# Autodesk Inventor assembly: Full_SigmaBan_106AT_nuc
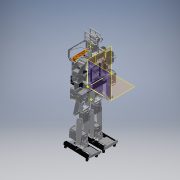
[picture p0: Inventor's stored thumbnail of the model, 180x180]
Saved by Autodesk Inventor 2018 (Build 220112000, 112)
## iProperties
Created: 2017-01-31
Part Number: Full_SigmaBan_106AT_nuc
Document SubType Name: Assembly
Designer: steve
Mass: 4494.03 g
Surface Area: 10713.9 cm^2
Volume: 2303.92 cm^3
Density: 1.9506 g/cm^3
Author: steve
## Documents named in this file (44)
- C:\Users\patxi\Dropbox\SigmaBan\SigmaBanV2.1\Full_SigmaBan_106AT_nuc.iam
- C:\Users\patxi\Dropbox\SigmaBan\SigmaBanV2.1\SigmaBan_torsebas64.ipt
- C:\Users\patxi\Dropbox\SigmaBan\SigmaBanV2.1\battery.ipt
- C:\Users\patxi\Dropbox\SigmaBan\SigmaBanV2.1\backboard.ipt
- C:\Users\patxi\Dropbox\SigmaBan\SigmaBanV2.1\newhub.ipt
- C:\Users\patxi\Dropbox\SigmaBan\SigmaBanV2.1\MX-64AT_AR_sideR.iam
- C:\Users\patxi\Dropbox\SigmaBan\SigmaBanV2.1\MX-64AT_AR_sideL.iam
- C:\Users\patxi\Dropbox\SigmaBan\SigmaBanV2.1\bloc_double106.iam
- C:\Users\patxi\Dropbox\SigmaBan\SigmaBanV2.1\MX-106T_bottom.iam
- C:\Users\patxi\Dropbox\SigmaBan\SigmaBanV2.1\Sigma106_tibiaplate_design.ipt
- C:\Users\patxi\Dropbox\SigmaBan\SigmaBanV2.1\MX-64AT_AR_contreaxe.iam
- C:\Users\patxi\Dropbox\SigmaBan\SigmaBanV2.1\beeper.ipt
- C:\Users\patxi\Dropbox\SigmaBan\SigmaBanV2.1\pillar_tube.ipt
- C:\Users\patxi\Dropbox\SigmaBan\SigmaBanV2.1\fitplate.ipt
- C:\Users\patxi\Dropbox\SigmaBan\SigmaBanV2.1\new_torso_topplate_nuc.ipt
- C:\Users\patxi\Dropbox\SigmaBan\SigmaBanV2.1\new_torso_middleplate_nuc.ipt
- C:\Users\patxi\Dropbox\SigmaBan\SigmaBanV2.1\Intel NUC6i3SYK.ipt
- C:\Users\patxi\Dropbox\SigmaBan\SigmaBanV2.1\new_U\new_u64_2.iam
- C:\Users\patxi\Dropbox\SigmaBan\SigmaBanV2.1\Ulong\u106_long_design_newbearing.iam
- C:\Users\patxi\Dropbox\SigmaBan\SigmaBanV2.1\piano_wire_protection.ipt
- C:\Users\patxi\Dropbox\SigmaBan\SigmaBanV2.1\high_leg_teflon_left.ipt
- C:\Users\patxi\Dropbox\SigmaBan\SigmaBanV2.1\high_leg_teflon_right.ipt
- C:\Users\patxi\Dropbox\SigmaBan\SigmaBanV2.1\new_U\new_U64_shoulder_with_offset.iam
- C:\Users\patxi\Dropbox\SigmaBan\SigmaBanV2.1\humerus.ipt
- C:\Users\patxi\Dropbox\SigmaBan\SigmaBanV2.1\FR05-H101.ipt
- C:\Users\patxi\Dropbox\SigmaBan\SigmaBanV2.1\FR05-S101.ipt
- C:\Users\patxi\Dropbox\SigmaBan\SigmaBanV2.1\radius.ipt
- C:\Users\patxi\Dropbox\SigmaBan\SigmaBanV2.1\elbow_protection.ipt
- C:\Users\patxi\Dropbox\SigmaBan\SigmaBanV2.1\new_u64_shoulder.iam
- C:\Users\patxi\Dropbox\SigmaBan\SigmaBanV2.1\head_mx64\head_assembly.iam
- C:\Users\patxi\Dropbox\SigmaBan\SigmaBanV2.1\nuc_fix_v2.ipt
- C:\Users\patxi\Dropbox\SigmaBan\SigmaBanV2.1\piano_wire_back_fixation.ipt
- C:\Users\patxi\Dropbox\SigmaBan\SigmaBanV2.1\back_piano_wire.ipt
- C:\Users\patxi\Dropbox\SigmaBan\SigmaBanV2.1\shoulder_piano_wire_fix.ipt
- C:\Users\patxi\Dropbox\SigmaBan\SigmaBanV2.1\shoulder_piano wire.ipt
- C:\Users\patxi\Dropbox\SigmaBan\SigmaBanV2.1\foot_with_cleat.iam
- C:\Users\patxi\Dropbox\SigmaBan\SigmaBanV2.1\bloc_double106_MIR.iam
- C:\Users\patxi\Dropbox\SigmaBan\SigmaBanV2.1\dynamixel\frames\FR08-B101.ipt
- C:\Users\patxi\Dropbox\SigmaBan\SigmaBanV2.1\MX-64AT_AR.ipt
- C:\Users\patxi\Dropbox\SigmaBan\SigmaBanV2.1\dynamixel\motors\mx106-contre-axe.iam
- C:\Users\patxi\Dropbox\SigmaBan\SigmaBanV2.1\low_torso_protection.ipt
- C:\Users\patxi\Dropbox\SigmaBan\SigmaBanV2.1\high_torso_protection.ipt
- C:\Users\patxi\Dropbox\SigmaBan\SigmaBanV2.1\external\M3_cube_standoff.ipt
- C:\Users\patxi\Dropbox\SigmaBan\SigmaBanV2.1\handle_v3.ipt
## Components (80 placed, 49 different names)
1. SigmaBan_torsebas64:1 — Mate:98, Flush:8, Flush:9, Mate:548, Mate:551, Mate:552, Mate:553
2. FR08-B101:1 — Mate:442, Mate:443, Mate:481, Mate:482, Mate:483
3. FR08-B101:2 — Mate:446, Mate:447, Mate:448, Mate:473, Mate:474, Mate:475
4. battery:1 — Mate:98, Flush:8, Flush:9
5. new_torso_topplate_nuc:1 — Mate:57, Mate:58, Mate:59, Mate:60, Mate:61, Mate:62, Mate:233, Mate:234, Mate:235, Mate:248, Mate:249, Mate:251, Flush:3, Mate:252, Mate:271, Flush:5, Mate:391, Mate:392, Mate:453, Mate:456, Flush:11, Mate:555, Flush:12, Mate:556, Mate:560, Mate:561, Mate:562, Mate:564, Mate:565, Mate:566
6. new_torso_middleplate_nuc:1 — Mate:214, Mate:215, Mate:236, Mate:239, Mate:240, Mate:241, Mate:242, Mate:256, Mate:257, Mate:258, Mate:259, Flush:4, Mate:442, Mate:443, Mate:446, Mate:447, Mate:448, Mate:550, Mate:554
7. Motor:right_shoulder_pitch [sub-assembly] — Mate:57, Mate:59, Mate:60, Mate:349, Mate:350
8. Motor:left_shoulder_pitch [sub-assembly] — Mate:58, Mate:61, Mate:62, Mate:345, Mate:346, DOF:left_shoulder_pitch
9. Motor:right_hip_pitch — Mate:473, Mate:474, Mate:475, Mate:476, Mate:477, Mate:478, Mate:479, Mate:480, Mate:551, Mate:552, Mate:553
10. Motor:left_hip [sub-assembly] — Mate:141, Mate:282, Mate:428, Mate:539, Mate:540, DOF:left_hip_pitch, DOF:left_hip_yaw, DOF:left_hip_roll
11. Motor:right_hip [sub-assembly] — Mate:278, Mate:435, Mate:541, Mate:542
12. Motor:left_knee [sub-assembly] — Mate:150, Mate:164, Mate:287, DOF:left_hip_pitch, DOF:left_knee, Mate:429, Mate:430, Mate:431, Mate:432
13. Motor:left_ankle [sub-assembly] — Mate:143, Mate:151, Mate:162, Mate:163, DOF:left_ankle_pitch, Mate:543, Mate:544
14. Motor:right_ankle [sub-assembly] — DOF:right_ankle_pitch, Mate:433, Mate:434, Mate:439, Mate:545, Mate:546
15. Sigma106_tibiaplate_design:1 — Mate:150, Mate:151, DOF:left_knee, DOF:left_ankle_pitch, Mate:432
16. Sigma106_tibiaplate_design:2 — DOF:right_ankle_pitch, Mate:433, Mate:434, Mate:464, Mate:466
17. Sigma106_tibiaplate_design:3 — Mate:439, Mate:465, Mate:547
18. Sigma106_tibiaplate_design:4 — Mate:162, Mate:163, Mate:164, Mate:431
19. u106_long_design_newbearing:1 [sub-assembly] — Mate:282, Mate:287, Mate:428, Mate:429, Mate:430
20. u106_long_design_newbearing:2 [sub-assembly] — Mate:278, Mate:435, Mate:470, Mate:471, Mate:472
21. new_u64_2:2 [sub-assembly] — Mate:484, Mate:485, Mate:539, Mate:540
22. new_u64_2:3 [sub-assembly] — Mate:416, Mate:417, Mate:418, Mate:543, Mate:544
23. new_u64_2:4 [sub-assembly] — Mate:476, Mate:477, Mate:541, Mate:542
24. new_u64_2:5 [sub-assembly] — Mate:421, Mate:422, Mate:423, Mate:545, Mate:546
25. Motor:left_shoulder_roll [sub-assembly] — Mate:347, Mate:348, Mate:404, Mate:405, Mate:406, Mate:407, Mate:408, Mate:409, DOF:left_shoulder_roll, Mate:491, Mate:492, Mate:493
26. newhub:2 — Mate:214, Mate:215, Mate:441, Flush:10
27. backboard:3 — Mate:233, Mate:234, Mate:235
28. beeper:1 — Mate:236, Mate:441, Flush:10
29. pillar_tube:1 — Mate:239, Mate:248, Mate:256
30. pillar_tube:2 — Mate:240, Mate:249, Mate:259
31. pillar_tube:3 — Mate:242, Mate:258, Mate:390
32. pillar_tube:4 — Mate:241, Mate:257, Mate:271
33. fitplate:1 — Mate:251, Flush:3, Mate:252
34. MX-64AT_AR_contreaxe:2 [sub-assembly] — Mate:351, Mate:352, Angle:29, Mate:503, Mate:504, Mate:505, Mate:534, Mate:535, Mate:536
35. Intel NUC6i3SYK:1 — Flush:4, Flush:5, Flush:11
36. FR08-B101:3 — Mate:453, Mate:456, Mate:458, Mate:460, Mate:461
37. piano_wire_protection:1 — Mate:563, Mate:567
38. high_leg_teflon_left:1 — Mate:486, Mate:487, Mate:488
39. high_leg_teflon_right:1 — Mate:478, Mate:479, Mate:480
40. new_U64_shoulder_with_offset:1 [sub-assembly] — Mate:345, Mate:346, Mate:347, Mate:348, DOF:left_shoulder_pitch, DOF:left_shoulder_roll
41. new_U64_shoulder_with_offset:2 [sub-assembly] — Mate:349, Mate:350, Mate:351, Mate:352, Angle:29
42. humerus:1 — Mate:372, Mate:373, Mate:374, DOF:left_elbow, Mate:494, Mate:495, Mate:496
43. humerus:2 — Mate:506, Mate:507, Mate:508, Mate:519, Mate:520, Mate:521
44. FR05-H101:1 — Mate:372, Mate:373, Mate:374, Mate:375, Mate:376, Mate:383, Mate:384, Mate:385
45. Motor:left_elbow [sub-assembly] — Mate:375, Mate:376, DOF:left_elbow, Mate:497, Mate:498, Mate:499
46. FR05-S101:1 — Mate:497, Mate:498, Mate:499, Mate:500, Mate:501, Mate:502
47. radius:1 — Mate:500, Mate:501, Mate:502
48. elbow_protection:1 — Mate:383, Mate:384, Mate:385
49. new_u64_shoulder:1 [sub-assembly] — DOF:head_pitch, Mate:413, Mate:414, Mate:457, Mate:459
50. head_assembly:1 [sub-assembly] — DOF:head_pitch, Mate:413, Mate:414, DOF:head_yaw
51. nuc_fix_v2:1 — Mate:390, Mate:391, Mate:392, Mate:393, Mate:394, Mate:395, Mate:396, Mate:397, Mate:398
52. piano_wire_back_fixation:1 — Mate:393, Mate:394, Mate:395, Mate:400, Mate:570, Mate:571
53. piano_wire_back_fixation:2 — Mate:396, Mate:397, Mate:398, Mate:399, Mate:401, Mate:568, Mate:569
54. back_piano_wire:1 — Mate:399, Mate:400, Mate:401
55. shoulder_piano_wire_fix:1 — Mate:404, Mate:405, Mate:406, Mate:411, Mate:412
56. shoulder_piano_wire_fix:2 — Mate:407, Mate:408, Mate:409, Mate:410
57. shoulder_piano wire:1 — Mate:410, Mate:411, Mate:412
58. foot_with_cleat:1 [sub-assembly] — Mate:416, Mate:417, Mate:418
59. foot_with_cleat:2 [sub-assembly] — Mate:421, Mate:422, Mate:423
60. Motor:head_yaw — Mate:457, Mate:458, Mate:459, Mate:460, Mate:461, DOF:head_yaw, Flush:13
61. mx106-contre-axe:1 [sub-assembly] — Mate:464, Mate:465, Mate:466, Mate:467, Mate:468, Mate:469, Mate:547
62. FR05-S101:2 — Mate:467, Mate:468, Mate:469, Mate:470, Mate:471, Mate:472
63. Motor:left_hip_yaw — Mate:481, Mate:482, Mate:483, Mate:484, Mate:485, Mate:486, Mate:487, Mate:488, DOF:left_hip_yaw, DOF:left_hip_roll
64. FR05-S101:3 — Mate:491, Mate:492, Mate:493, Mate:494, Mate:495, Mate:496
65. FR05-S101:4 — Mate:503, Mate:504, Mate:505, Mate:506, Mate:507, Mate:508
66. FR05-H101:2 — Mate:517, Mate:518, Mate:519, Mate:520, Mate:521, Mate:525, Mate:526, Mate:527
67. MX-64AT_AR_contreaxe:4 [sub-assembly] — Mate:517, Mate:518, Mate:522, Mate:523, Mate:524
68. FR05-S101:5 — Mate:522, Mate:523, Mate:524
69. radius:2
70. elbow_protection:2 — Mate:525, Mate:526, Mate:527
71. shoulder_piano_wire_fix:3 — Mate:532, Mate:533, Mate:534, Mate:535, Mate:536
72. shoulder_piano_wire_fix:4 — Mate:537, Mate:538
73. shoulder_piano wire:2 — Mate:532, Mate:533, Mate:537, Mate:538
74. low_torso_protection:1 — Mate:548, Mate:550, Mate:554
75. high_torso_protection:1 — Mate:555, Flush:12, Mate:556
76. piano_wire_back_fixation:3 — Mate:560, Mate:561, Mate:562, Mate:563, Mate:567
77. piano_wire_back_fixation:4 — Mate:564, Mate:565, Mate:566
78. M3_cube_standoff:1 — Mate:570, Mate:571, Mate:574
79. M3_cube_standoff:2 — Mate:568, Mate:569, Mate:572, Mate:573
80. handle_v3:1 — Mate:572, Mate:573, Mate:574
## Relationships (222: Mate 201, Angle 12, Flush 9)
- Mate:57: new_torso_topplate_nuc:1 ↔ Motor:right_shoulder_pitch
- Mate:58: new_torso_topplate_nuc:1 ↔ Motor:left_shoulder_pitch
- Mate:59: new_torso_topplate_nuc:1 ↔ Motor:right_shoulder_pitch
- Mate:60: new_torso_topplate_nuc:1 ↔ Motor:right_shoulder_pitch
- Mate:61: new_torso_topplate_nuc:1 ↔ Motor:left_shoulder_pitch
- Mate:62: new_torso_topplate_nuc:1 ↔ Motor:left_shoulder_pitch
- [Mate]: FR08-B101:1 ↔ new_torso_middleplate_nuc:1
- Mate:98: SigmaBan_torsebas64:1 ↔ battery:1
- Mate:141: Motor:left_hip
- Mate:143: Motor:left_ankle
- Mate:150: Motor:left_knee ↔ Sigma106_tibiaplate_design:1
- Mate:151: Motor:left_ankle ↔ Sigma106_tibiaplate_design:1
- Mate:162: Motor:left_ankle ↔ Sigma106_tibiaplate_design:4
- Mate:163: Motor:left_ankle ↔ Sigma106_tibiaplate_design:4
- Mate:164: Motor:left_knee ↔ Sigma106_tibiaplate_design:4
- Mate:214: new_torso_middleplate_nuc:1 ↔ newhub:2
- Mate:215: new_torso_middleplate_nuc:1 ↔ newhub:2
- Mate:233: new_torso_topplate_nuc:1 ↔ backboard:3
- Mate:234: new_torso_topplate_nuc:1 ↔ backboard:3
- Mate:235: new_torso_topplate_nuc:1 ↔ backboard:3
- Mate:236: new_torso_middleplate_nuc:1 ↔ beeper:1
- Mate:239: new_torso_middleplate_nuc:1 ↔ pillar_tube:1
- Mate:240: new_torso_middleplate_nuc:1 ↔ pillar_tube:2
- Mate:241: new_torso_middleplate_nuc:1 ↔ pillar_tube:4
- Mate:242: new_torso_middleplate_nuc:1 ↔ pillar_tube:3
- Mate:248: new_torso_topplate_nuc:1 ↔ pillar_tube:1
- Mate:249: new_torso_topplate_nuc:1 ↔ pillar_tube:2
- Mate:251: new_torso_topplate_nuc:1 ↔ fitplate:1
- Flush:3: new_torso_topplate_nuc:1 ↔ fitplate:1
- Mate:252: new_torso_topplate_nuc:1 ↔ fitplate:1
- Mate:256: new_torso_middleplate_nuc:1 ↔ pillar_tube:1
- Mate:257: new_torso_middleplate_nuc:1 ↔ pillar_tube:4
- Mate:258: new_torso_middleplate_nuc:1 ↔ pillar_tube:3
- Mate:259: new_torso_middleplate_nuc:1 ↔ pillar_tube:2
- Mate:271: new_torso_topplate_nuc:1 ↔ pillar_tube:4
- Flush:4: new_torso_middleplate_nuc:1 ↔ Intel NUC6i3SYK:1
- Flush:5: new_torso_topplate_nuc:1 ↔ Intel NUC6i3SYK:1
- Mate:278: Motor:right_hip ↔ u106_long_design_newbearing:2
- Mate:282: Motor:left_hip ↔ u106_long_design_newbearing:1
- Mate:287: Motor:left_knee ↔ u106_long_design_newbearing:1
- [Mate]: new_torso_topplate_nuc:1 ↔ FR08-B101:3
- Flush:8: SigmaBan_torsebas64:1 ↔ battery:1
- Flush:9: SigmaBan_torsebas64:1 ↔ battery:1
- Mate:345: Motor:left_shoulder_pitch ↔ new_U64_shoulder_with_offset:1
- Mate:346: Motor:left_shoulder_pitch ↔ new_U64_shoulder_with_offset:1
- Mate:347: Motor:left_shoulder_roll ↔ new_U64_shoulder_with_offset:1
- Mate:348: Motor:left_shoulder_roll ↔ new_U64_shoulder_with_offset:1
- Mate:349: Motor:right_shoulder_pitch ↔ new_U64_shoulder_with_offset:2
- Mate:350: Motor:right_shoulder_pitch ↔ new_U64_shoulder_with_offset:2
- Mate:351: MX-64AT_AR_contreaxe:2 ↔ new_U64_shoulder_with_offset:2
- Mate:352: MX-64AT_AR_contreaxe:2 ↔ new_U64_shoulder_with_offset:2
- Angle:29 (0 deg): MX-64AT_AR_contreaxe:2 ↔ new_U64_shoulder_with_offset:2
- Mate:372: humerus:1 ↔ FR05-H101:1
- Mate:373: humerus:1 ↔ FR05-H101:1
- Mate:374: humerus:1 ↔ FR05-H101:1
- Mate:375: FR05-H101:1 ↔ Motor:left_elbow
- Mate:376: FR05-H101:1 ↔ Motor:left_elbow
- DOF:left_elbow [Angle] (0 deg): humerus:1 ↔ Motor:left_elbow
- Mate:383: FR05-H101:1 ↔ elbow_protection:1
- Mate:384: FR05-H101:1 ↔ elbow_protection:1
- Mate:385: FR05-H101:1 ↔ elbow_protection:1
- DOF:head_pitch [Angle] (0 deg): new_u64_shoulder:1 ↔ head_assembly:1
- Mate:390: pillar_tube:3 ↔ nuc_fix_v2:1
- Mate:391: new_torso_topplate_nuc:1 ↔ nuc_fix_v2:1
- Mate:392: new_torso_topplate_nuc:1 ↔ nuc_fix_v2:1
- Mate:393: nuc_fix_v2:1 ↔ piano_wire_back_fixation:1
- Mate:394: nuc_fix_v2:1 ↔ piano_wire_back_fixation:1
- Mate:395: nuc_fix_v2:1 ↔ piano_wire_back_fixation:1
- Mate:396: nuc_fix_v2:1 ↔ piano_wire_back_fixation:2
- Mate:397: nuc_fix_v2:1 ↔ piano_wire_back_fixation:2
- Mate:398: nuc_fix_v2:1 ↔ piano_wire_back_fixation:2
- Mate:399: piano_wire_back_fixation:2 ↔ back_piano_wire:1
- Mate:400: piano_wire_back_fixation:1 ↔ back_piano_wire:1
- Mate:401: piano_wire_back_fixation:2 ↔ back_piano_wire:1
- Mate:404: Motor:left_shoulder_roll ↔ shoulder_piano_wire_fix:1
- Mate:405: Motor:left_shoulder_roll ↔ shoulder_piano_wire_fix:1
- Mate:406: Motor:left_shoulder_roll ↔ shoulder_piano_wire_fix:1
- Mate:407: Motor:left_shoulder_roll ↔ shoulder_piano_wire_fix:2
- Mate:408: Motor:left_shoulder_roll ↔ shoulder_piano_wire_fix:2
- Mate:409: Motor:left_shoulder_roll ↔ shoulder_piano_wire_fix:2
- Mate:410: shoulder_piano_wire_fix:2 ↔ shoulder_piano wire:1
- Mate:411: shoulder_piano_wire_fix:1 ↔ shoulder_piano wire:1
- Mate:412: shoulder_piano_wire_fix:1 ↔ shoulder_piano wire:1
- Mate:413: new_u64_shoulder:1 ↔ head_assembly:1
- Mate:414: new_u64_shoulder:1 ↔ head_assembly:1
- DOF:left_hip_pitch [Angle] (0 deg): Motor:left_hip ↔ Motor:left_knee
- DOF:left_knee [Angle] (0 deg): Motor:left_knee ↔ Sigma106_tibiaplate_design:1
- DOF:left_ankle_pitch [Angle] (0 deg): Motor:left_ankle ↔ Sigma106_tibiaplate_design:1
- DOF:left_shoulder_pitch [Angle] (0 deg): Motor:left_shoulder_pitch ↔ new_U64_shoulder_with_offset:1
- DOF:left_shoulder_roll [Angle] (0 deg): Motor:left_shoulder_roll ↔ new_U64_shoulder_with_offset:1
- Mate:416: new_u64_2:3 ↔ foot_with_cleat:1
- Mate:417: new_u64_2:3 ↔ foot_with_cleat:1
- Mate:418: new_u64_2:3 ↔ foot_with_cleat:1
- Mate:421: new_u64_2:5 ↔ foot_with_cleat:2
- Mate:422: new_u64_2:5 ↔ foot_with_cleat:2
- DOF:right_ankle_pitch [Angle] (0 deg): Motor:right_ankle ↔ Sigma106_tibiaplate_design:2
- Mate:423: new_u64_2:5 ↔ foot_with_cleat:2
- Mate:428: Motor:left_hip ↔ u106_long_design_newbearing:1
- Mate:429: Motor:left_knee ↔ u106_long_design_newbearing:1
- Mate:430: Motor:left_knee ↔ u106_long_design_newbearing:1
- Mate:431: Motor:left_knee ↔ Sigma106_tibiaplate_design:4
- Mate:432: Motor:left_knee ↔ Sigma106_tibiaplate_design:1
- Mate:433: Motor:right_ankle ↔ Sigma106_tibiaplate_design:2
- Mate:434: Motor:right_ankle ↔ Sigma106_tibiaplate_design:2
- Mate:435: Motor:right_hip ↔ u106_long_design_newbearing:2
- Mate:439: Motor:right_ankle ↔ Sigma106_tibiaplate_design:3
- Mate:441: newhub:2 ↔ beeper:1
- Flush:10: newhub:2 ↔ beeper:1
- Mate:442: FR08-B101:1 ↔ new_torso_middleplate_nuc:1
- Mate:443: FR08-B101:1 ↔ new_torso_middleplate_nuc:1
- Mate:446: FR08-B101:2 ↔ new_torso_middleplate_nuc:1
- Mate:447: FR08-B101:2 ↔ new_torso_middleplate_nuc:1
- Mate:448: FR08-B101:2 ↔ new_torso_middleplate_nuc:1
- Mate:453: new_torso_topplate_nuc:1 ↔ FR08-B101:3
- Mate:456: new_torso_topplate_nuc:1 ↔ FR08-B101:3
- Mate:457: new_u64_shoulder:1 ↔ Motor:head_yaw
- Mate:458: FR08-B101:3 ↔ Motor:head_yaw
- Mate:459: new_u64_shoulder:1 ↔ Motor:head_yaw
- Mate:460: FR08-B101:3 ↔ Motor:head_yaw
- Mate:461: FR08-B101:3 ↔ Motor:head_yaw
- Mate:464: Sigma106_tibiaplate_design:2 ↔ mx106-contre-axe:1
- Mate:465: Sigma106_tibiaplate_design:3 ↔ mx106-contre-axe:1
- Mate:466: Sigma106_tibiaplate_design:2 ↔ mx106-contre-axe:1
- Mate:467: mx106-contre-axe:1 ↔ FR05-S101:2
- Mate:468: mx106-contre-axe:1 ↔ FR05-S101:2
- Mate:469: mx106-contre-axe:1 ↔ FR05-S101:2
- Mate:470: u106_long_design_newbearing:2 ↔ FR05-S101:2
- Mate:471: u106_long_design_newbearing:2 ↔ FR05-S101:2
- Mate:472: u106_long_design_newbearing:2 ↔ FR05-S101:2
- Mate:473: FR08-B101:2 ↔ Motor:right_hip_pitch
- Mate:474: FR08-B101:2 ↔ Motor:right_hip_pitch
- Mate:475: FR08-B101:2 ↔ Motor:right_hip_pitch
- Mate:476: Motor:right_hip_pitch ↔ new_u64_2:4
- Mate:477: Motor:right_hip_pitch ↔ new_u64_2:4
- Mate:478: Motor:right_hip_pitch ↔ high_leg_teflon_right:1
- Mate:479: Motor:right_hip_pitch ↔ high_leg_teflon_right:1
- Mate:480: Motor:right_hip_pitch ↔ high_leg_teflon_right:1
- Mate:481: FR08-B101:1 ↔ Motor:left_hip_yaw
- Mate:482: FR08-B101:1 ↔ Motor:left_hip_yaw
- Mate:483: FR08-B101:1 ↔ Motor:left_hip_yaw
- Mate:484: new_u64_2:2 ↔ Motor:left_hip_yaw
- Mate:485: new_u64_2:2 ↔ Motor:left_hip_yaw
- Mate:486: high_leg_teflon_left:1 ↔ Motor:left_hip_yaw
- Mate:487: high_leg_teflon_left:1 ↔ Motor:left_hip_yaw
- Mate:488: high_leg_teflon_left:1 ↔ Motor:left_hip_yaw
- Mate:491: Motor:left_shoulder_roll ↔ FR05-S101:3
- Mate:492: Motor:left_shoulder_roll ↔ FR05-S101:3
- Mate:493: Motor:left_shoulder_roll ↔ FR05-S101:3
- Mate:494: humerus:1 ↔ FR05-S101:3
- Mate:495: humerus:1 ↔ FR05-S101:3
- Mate:496: humerus:1 ↔ FR05-S101:3
- Mate:497: Motor:left_elbow ↔ FR05-S101:1
- Mate:498: Motor:left_elbow ↔ FR05-S101:1
- Mate:499: Motor:left_elbow ↔ FR05-S101:1
- Mate:500: FR05-S101:1 ↔ radius:1
- Mate:501: FR05-S101:1 ↔ radius:1
- Mate:502: FR05-S101:1 ↔ radius:1
- Mate:503: MX-64AT_AR_contreaxe:2 ↔ FR05-S101:4
- Mate:504: MX-64AT_AR_contreaxe:2 ↔ FR05-S101:4
- Mate:505: MX-64AT_AR_contreaxe:2 ↔ FR05-S101:4
- Mate:506: humerus:2 ↔ FR05-S101:4
- Mate:507: humerus:2 ↔ FR05-S101:4
- Mate:508: humerus:2 ↔ FR05-S101:4
- [Mate]: FR05-S101:5 ↔ radius:2
- [Mate]: FR05-S101:5 ↔ radius:2
- [Mate]: FR05-S101:5 ↔ radius:2
- Mate:517: FR05-H101:2 ↔ MX-64AT_AR_contreaxe:4
- Mate:518: FR05-H101:2 ↔ MX-64AT_AR_contreaxe:4
- Mate:519: humerus:2 ↔ FR05-H101:2
- Mate:520: humerus:2 ↔ FR05-H101:2
- Mate:521: humerus:2 ↔ FR05-H101:2
- Mate:522: MX-64AT_AR_contreaxe:4 ↔ FR05-S101:5
- Mate:523: MX-64AT_AR_contreaxe:4 ↔ FR05-S101:5
- Mate:524: MX-64AT_AR_contreaxe:4 ↔ FR05-S101:5
- Mate:525: FR05-H101:2 ↔ elbow_protection:2
- Mate:526: FR05-H101:2 ↔ elbow_protection:2
- Mate:527: FR05-H101:2 ↔ elbow_protection:2
- Mate:532: shoulder_piano_wire_fix:3 ↔ shoulder_piano wire:2
- Mate:533: shoulder_piano_wire_fix:3 ↔ shoulder_piano wire:2
- Mate:534: MX-64AT_AR_contreaxe:2 ↔ shoulder_piano_wire_fix:3
- Mate:535: MX-64AT_AR_contreaxe:2 ↔ shoulder_piano_wire_fix:3
- Mate:536: MX-64AT_AR_contreaxe:2 ↔ shoulder_piano_wire_fix:3
- Mate:537: shoulder_piano_wire_fix:4 ↔ shoulder_piano wire:2
- Mate:538: shoulder_piano_wire_fix:4 ↔ shoulder_piano wire:2
- Mate:539: Motor:left_hip ↔ new_u64_2:2
- Mate:540: Motor:left_hip ↔ new_u64_2:2
- Mate:541: Motor:right_hip ↔ new_u64_2:4
- Mate:542: Motor:right_hip ↔ new_u64_2:4
- Mate:543: Motor:left_ankle ↔ new_u64_2:3
- Mate:544: Motor:left_ankle ↔ new_u64_2:3
- Mate:545: Motor:right_ankle ↔ new_u64_2:5
- Mate:546: Motor:right_ankle ↔ new_u64_2:5
- Mate:547: Sigma106_tibiaplate_design:3 ↔ mx106-contre-axe:1
- Mate:548: SigmaBan_torsebas64:1 ↔ low_torso_protection:1
- Flush:11: new_torso_topplate_nuc:1 ↔ Intel NUC6i3SYK:1
- Mate:550: new_torso_middleplate_nuc:1 ↔ low_torso_protection:1
- Mate:551: SigmaBan_torsebas64:1 ↔ Motor:right_hip_pitch
- Mate:552: SigmaBan_torsebas64:1 ↔ Motor:right_hip_pitch
- Mate:553: SigmaBan_torsebas64:1 ↔ Motor:right_hip_pitch
- Mate:554: new_torso_middleplate_nuc:1 ↔ low_torso_protection:1
- Mate:555: new_torso_topplate_nuc:1 ↔ high_torso_protection:1
- Flush:12: new_torso_topplate_nuc:1 ↔ high_torso_protection:1
- Mate:556: new_torso_topplate_nuc:1 ↔ high_torso_protection:1
- Mate:560: new_torso_topplate_nuc:1 ↔ piano_wire_back_fixation:3
- Mate:561: new_torso_topplate_nuc:1 ↔ piano_wire_back_fixation:3
- Mate:562: new_torso_topplate_nuc:1 ↔ piano_wire_back_fixation:3
- Mate:563: piano_wire_protection:1 ↔ piano_wire_back_fixation:3
- Mate:564: new_torso_topplate_nuc:1 ↔ piano_wire_back_fixation:4
- Mate:565: new_torso_topplate_nuc:1 ↔ piano_wire_back_fixation:4
- Mate:566: new_torso_topplate_nuc:1 ↔ piano_wire_back_fixation:4
- Mate:567: piano_wire_protection:1 ↔ piano_wire_back_fixation:3
- Mate:568: piano_wire_back_fixation:2 ↔ M3_cube_standoff:2
- Mate:569: piano_wire_back_fixation:2 ↔ M3_cube_standoff:2
- Mate:570: piano_wire_back_fixation:1 ↔ M3_cube_standoff:1
- Mate:571: piano_wire_back_fixation:1 ↔ M3_cube_standoff:1
- Mate:572: M3_cube_standoff:2 ↔ handle_v3:1
- Mate:573: M3_cube_standoff:2 ↔ handle_v3:1
- Mate:574: M3_cube_standoff:1 ↔ handle_v3:1
- DOF:left_hip_yaw [Angle] (0 deg): Motor:left_hip ↔ Motor:left_hip_yaw
- DOF:left_hip_roll [Angle] (0 deg): Motor:left_hip ↔ Motor:left_hip_yaw
- DOF:head_yaw [Angle] (0 deg): head_assembly:1 ↔ Motor:head_yaw
- Flush:13: Motor:head_yaw
## Named parameters: d717_d703 = 0 mm, d718_d704 = 0 mm, d719_d705 = 0 mm
